# Autodesk Inventor assembly: Assembly1
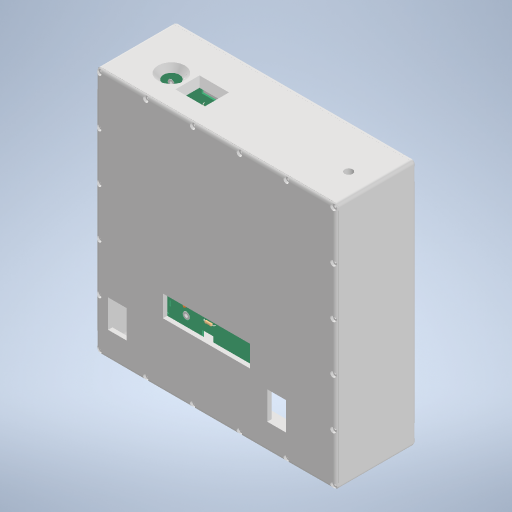
[picture p0: Inventor's stored thumbnail of the model, 512x512]
Saved by Autodesk Inventor 2024 (Build 280153000, 153)
## iProperties
Created: 2023-05-26
Part Number: Assembly1
Document SubType Name: Assembly
Designer: elect
Author: elect
## Documents named in this file (5)
- C:\Users\elect\JDC\Electronics\Projects\righteous_tentacle_colecovision\models\inventor_2024\Assembly1.iam
- C:\Users\elect\JDC\Electronics\Projects\righteous_tentacle_colecovision\models\inventor_2024\base_case\bottom.ipt
- C:\Users\elect\JDC\Electronics\Projects\righteous_tentacle_colecovision\models\FreeCAD\MainBoard\main_exports_missing-coleco_original_main_only\main_exports_missing-coleco_original_main_only.iam
- C:\Users\elect\JDC\Electronics\Projects\righteous_tentacle_colecovision\models\inventor_2024\base_case\middle.ipt
- C:\Users\elect\JDC\Electronics\Projects\righteous_tentacle_colecovision\models\inventor_2024\base_case\top.ipt
## Components (4 placed, 4 different names)
1. bottom:1 — Mate:1, Mate:2
2. main_exports_missing-coleco_original_main_only:1 [sub-assembly] — Mate:1
3. middle:1 — Mate:2, Mate:3, Mate:4
4. top:1 — Mate:3, Mate:4
## Relationships (4: Mate 4)
- Mate:1: bottom:1 ↔ main_exports_missing-coleco_original_main_only:1
- Mate:2: bottom:1 ↔ middle:1
- Mate:3: middle:1 ↔ top:1
- Mate:4: middle:1 ↔ top:1
